# Autodesk Inventor assembly: !drivetrain
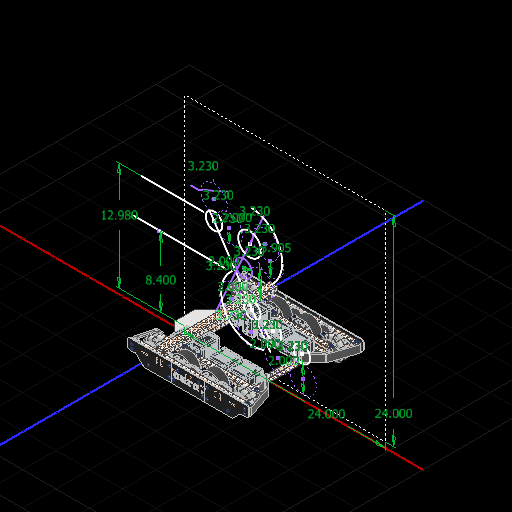
[picture p0: Inventor's stored thumbnail of the model, 512x512]
Saved by Autodesk Inventor 2025.2 (Build 292293000, 293)
## iProperties
Created: 2025-11-15
Part Number: !drivetrain
Document SubType Name: Assembly
Designer: cloudy
Mass: 2833.59 g
Surface Area: 13149.9 cm^2
Volume: 1429.88 cm^3
Density: 1.9817 g/cm^3
Author: cloudy
## Documents named in this file (40)
- C:\Users\cloudy\Documents\AURA_CAD\24\Drivetrain\!drivetrain.iam
- C:\Users\cloudy\Documents\AURA_CAD\24\Drivetrain\Wheels\Omni\2.75\2.75 Omni Assembly.iam
- C:\Users\cloudy\Documents\AURA_CAD\!lib\Structure\C Channel\Aluminum 1x2x1\Alu C 1x2x1x28.ipt
- C:\Users\cloudy\Documents\AURA_CAD\!lib\Structure\Hardware\Screw Steel - Star\SScrew Star Smooth 2.000.ipt
- C:\Users\cloudy\Documents\AURA_CAD\!lib\Structure\Hardware\Nut Keps.ipt
- C:\Users\cloudy\Documents\AURA_CAD\24\Drivetrain\Gears\26t_no_screwholes.ipt
- C:\Users\cloudy\Documents\AURA_CAD\!lib\Electronics\Motors with Screws\AluM-StarS.iam
- C:\Users\cloudy\Documents\AURA_CAD\24\Drivetrain\bearing_2 long.ipt
- C:\Users\cloudy\Documents\AURA_CAD\!lib\Motion\Spacers\Spacer Nylon .500 OD\NSpacer White .500 OD x .125.ipt
- C:\Users\cloudy\Documents\AURA_CAD\!lib\Motion\Spacers\Spacer Nylon .375 OD\NSpacer .375 OD x .500.ipt
- C:\Users\cloudy\Documents\AURA_CAD\!lib\Motion\Spacers\Spacer Nylon .375 OD\NSpacer .375 OD x .250.ipt
- C:\Users\cloudy\Documents\AURA_CAD\!lib\Motion\Shaft LS\Bearing Flat - Drilled.ipt
- C:\Users\cloudy\Documents\AURA_CAD\!lib\Motion\Shaft LS\Shaft Collar Metal\Shaft Collar No Screw.iam
- C:\Users\cloudy\Documents\AURA_CAD\!lib\Motion\Spacers\Spacer Nylon .375 OD\NSpacer .375 OD x .375.ipt
- C:\Users\cloudy\Documents\AURA_CAD\!lib\Structure\C Channel\Aluminum 1x3x1 Half\Alu C Half 1x3x1x3.ipt
- C:\Users\cloudy\Documents\AURA_CAD\24\Drivetrain\Wheels\Traction\traction.iam
- C:\Users\cloudy\Documents\AURA_CAD\!lib\Structure\Hardware\Nut Nylock.ipt
- C:\Users\cloudy\Documents\AURA_CAD\24\ziptie.ipt
- C:\Users\cloudy\Documents\AURA_CAD\!lib\Motion\Shaft LS\Shaft LS Capped\Shaft LS Capped 3.0.ipt
- C:\Users\cloudy\Documents\AURA_CAD\!lib\Structure\Hardware\Screw Steel - Star\SScrew Star Smooth .375.ipt
- C:\Users\cloudy\Documents\AURA_CAD\!lib\Structure\Hardware\Screw Steel - Star\SScrew Star Threaded .500.ipt
- C:\Users\cloudy\Documents\AURA_CAD\24\Drivetrain\funnel.ipt
- C:\Users\cloudy\Documents\AURA_CAD\!lib\Structure\C Channel\Aluminum 1x3x1 Half Thick Cut\Alu C Half Thick 1x3x1x20.ipt
- C:\Users\cloudy\Documents\AURA_CAD\!lib\Motion\Spacers\Spacer Nylon .375 OD\NSpacer .375 OD x .125.ipt
- C:\Users\cloudy\Documents\AURA_CAD\24\funnelFront.ipt
- C:\Users\cloudy\Documents\AURA_CAD\24\plate.ipt
- C:\Users\cloudy\Documents\AURA_CAD\!lib\Structure\Hardware\Screw Steel - Star\SScrew Star Smooth 1.250.ipt
- C:\Users\cloudy\Documents\GitHub\aura-cad\!lib\Structure\Hardware\Screw Steel - Star.ipt
- C:\Users\cloudy\Documents\GitHub\aura-cad\!lib\Electronics\Motors with Screws.iam
- C:\Users\cloudy\Documents\GitHub\aura-cad\!lib\Motion\Spacers\Spacer Nylon .500 OD.ipt
- C:\Users\cloudy\Documents\GitHub\aura-cad\!lib\Motion\Spacers\Spacer Nylon .375 OD.ipt
- C:\Users\cloudy\Documents\GitHub\aura-cad\!lib\Motion\Shaft LS\Shaft Collar Metal.iam
- C:\Users\cloudy\Documents\GitHub\aura-cad\!lib\Motion\Shaft LS\Shaft LS Capped.ipt
- C:\Users\cloudy\Documents\AURA_CAD\!lib\Structure\C Channel\Aluminum 1x2x1\Alu C 1x2x1x27.ipt
- C:\Users\cloudy\Documents\AURA_CAD\!lib\Structure\C Channel\Aluminum 1x3x1 Half\Alu C Half 1x3x1x27.ipt
- C:\Users\cloudy\Documents\AURA_CAD\!lib\Structure\C Channel\Aluminum 1x2x1\Alu C 1x2x1x19.ipt
- C:\Users\cloudy\Documents\AURA_CAD\24\back_funnel.ipt
- C:\Users\cloudy\Documents\AURA_CAD\!lib\Structure\C Channel\Aluminum 1x2x1\Alu C 1x2x1x25.ipt
- C:\Users\cloudy\Documents\AURA_CAD\24\wedge.ipt
- C:\Users\cloudy\Documents\AURA_CAD\!lib\Miscellaneous\iw_metal_02.bmp
## Components (186 placed, 32 different names)
1. Alu C 1x2x1x25:2 — Insert:10, Insert:19, Insert:20, Insert:36, Insert:40, Mate:22, Mate:23, Insert:41, Insert:42, Insert:43, Insert:47, Mate:24, Insert:51, Insert:90, Mate:37, Mate:38, Insert:117, Insert:122, Insert:123, Insert:163, Insert:164, Insert:165, Mate:92, Insert:313, Insert:315, Mate:100, Insert:337, Mate:102, Insert:338
2. SScrew Star Smooth 2.000:1 — Insert:10, Mate:26
3. 2.75 Omni Assembly:5 [sub-assembly] — Insert:46
4. SScrew Star Smooth 2.000:2 — Insert:20
5. SScrew Star Smooth 2.000:3 — Insert:19
6. 2.75 Omni Assembly:7 [sub-assembly] — Insert:44
7. 26t_no_screwholes:1 — Insert:52, Insert:56
8. 26t_no_screwholes:2 — Insert:53, Insert:55
9. 26t_no_screwholes:3 — Insert:54, Insert:57
10. Alu C 1x2x1x28:3 — Mate:26, Insert:52, Insert:53, Insert:54, Insert:58, Insert:59, Insert:60, Mate:27, Mate:28, Mate:29, Insert:61, Mate:30, Insert:62, Insert:63, Insert:64, Mate:31, Mate:32, Mate:33, Insert:124, Insert:125, Insert:127, Insert:128, Insert:129, Insert:130, Insert:131, Insert:132, Insert:133, Insert:134, Mate:49, Mate:50, Mate:51, Mate:52, Mate:53, Mate:54, Mate:55, Mate:56, Mate:57, Mate:58, Insert:135, Insert:136, Insert:137, Insert:138, Insert:283, Insert:284, Mate:93, Insert:294, Mate:95, Insert:297, Mate:97, Insert:314, Insert:316, Insert:335
11. AluM-StarS:1 [sub-assembly] — Insert:36, Mate:22
12. AluM-StarS:2 [sub-assembly] — Insert:40, Mate:23
13. AluM-StarS:3 [sub-assembly] — Insert:47, Mate:24
14. Nut Keps:1 — Insert:41, Insert:44
15. Nut Keps:2 — Insert:42, Insert:111
16. Nut Keps:3 — Insert:43, Insert:46
17. NSpacer White .500 OD x .125:2 — Insert:51
18. NSpacer .375 OD x .250:2 — Insert:56
19. NSpacer .375 OD x .250:3 — Insert:55
20. NSpacer .375 OD x .250:4 — Insert:57
21. bearing_2 long:3 — Insert:59, Mate:28
22. bearing_2 long:4 — Insert:61, Mate:30, Insert:112
23. bearing_2 long:5 — Insert:58, Mate:29
24. bearing_2 long:6 — Insert:60, Mate:27
25. Bearing Flat - Drilled:1 — Insert:62, Mate:33
26. Bearing Flat - Drilled:2 — Insert:64, Mate:31
27. Bearing Flat - Drilled:3 — Insert:63, Mate:32
28. Alu C Half 1x3x1x3:1 — Insert:90, Mate:37, Insert:91, Insert:147, Insert:148
29. AluM-StarS:7 [sub-assembly] — Insert:91, Mate:38
30. traction:1 [sub-assembly] — Insert:113
31. traction:2 [sub-assembly] — Insert:111, Insert:114
32. NSpacer .375 OD x .250:9 — Insert:112, Insert:113
33. Nut Nylock:1 — Insert:114
34. NSpacer .375 OD x .500:10 — Insert:116, Insert:117
35. NSpacer .375 OD x .375:11 — Insert:115
36. Shaft Collar No Screw:6 [sub-assembly] — Insert:115, Insert:116
37. NSpacer .375 OD x .500:12 — Insert:122
38. NSpacer .375 OD x .375:13
39. Shaft Collar No Screw:7 [sub-assembly]
40. NSpacer .375 OD x .500:14 — Insert:123
41. NSpacer .375 OD x .375:15
42. Shaft Collar No Screw:8 [sub-assembly]
43. ziptie:1 — Insert:125, Mate:56
44. ziptie:2 — Insert:127, Mate:57
45. ziptie:3 — Insert:128, Mate:55
46. ziptie:4 — Insert:124, Mate:58
47. ziptie:5 — Insert:129, Mate:53
48. ziptie:6 — Insert:130, Mate:54
49. ziptie:7 — Insert:131, Mate:52
50. ziptie:8 — Insert:133, Mate:50
51. ziptie:9 — Insert:132, Mate:51
52. ziptie:10 — Insert:134, Mate:49
53. Shaft LS Capped 3.0:1 — Insert:135
54. Shaft LS Capped 3.0:2 — Insert:136
55. Shaft LS Capped 3.0:3 — Insert:137
56. Shaft LS Capped 3.0:4 — Insert:138
57. NSpacer White .500 OD x .125:4
58. Nut Keps:5 — Insert:147
59. Nut Keps:6 — Insert:148
60. Nut Keps:7
61. SScrew Star Threaded .500:7 — Insert:164
62. SScrew Star Smooth .375:8 — Insert:163
63. SScrew Star Smooth .375:10 — Insert:165
64. Alu C 1x2x1x25:1 — Insert:172, Insert:173, Insert:174, Mate:60, Insert:178, Mate:61, Insert:179, Mate:62, Insert:180, Insert:182, Insert:183, Insert:185, Insert:186, Mate:71, Insert:204, Mate:72, Insert:213, Insert:216, Insert:219, Insert:252, Insert:253, Insert:263, Mate:91, Insert:317, Insert:319, Mate:99, Mate:100
65. SScrew Star Smooth 2.000:17 — Insert:172, Mate:59
66. 2.75 Omni Assembly:8 [sub-assembly] — Insert:184
67. SScrew Star Smooth 2.000:18 — Insert:173
68. SScrew Star Smooth 2.000:19 — Insert:174
69. 2.75 Omni Assembly:9 [sub-assembly] — Insert:181
70. 26t_no_screwholes:4 — Insert:177, Insert:187
71. 26t_no_screwholes:5 — Insert:176, Insert:188
72. 26t_no_screwholes:6 — Insert:175, Insert:189
73. Alu C 1x2x1x28:4 — Insert:175, Insert:176, Insert:177, Mate:59, Mate:63, Insert:190, Mate:64, Insert:191, Mate:65, Insert:192, Mate:66, Insert:193, Mate:67, Insert:194, Mate:68, Insert:195, Mate:69, Insert:196, Mate:75, Insert:222, Mate:76, Insert:223, Mate:77, Insert:224, Mate:78, Insert:225, Mate:79, Insert:226, Mate:80, Insert:227, Mate:81, Insert:228, Mate:82, Insert:229, Mate:83, Insert:230, Mate:84, Insert:231, Insert:232, Insert:233, Insert:234, Insert:235, Insert:282, Insert:285, Mate:94, Insert:295, Insert:296, Mate:96, Mate:98, Insert:318, Insert:320, Mate:103, Insert:339
74. AluM-StarS:8 [sub-assembly] — Mate:60, Insert:178
75. AluM-StarS:9 [sub-assembly] — Mate:61, Insert:179
76. AluM-StarS:10 [sub-assembly] — Mate:62, Insert:180
77. Nut Keps:11 — Insert:181, Insert:182
78. Nut Keps:12 — Insert:183, Insert:209
79. Nut Keps:13 — Insert:184, Insert:185
80. NSpacer White .500 OD x .125:6 — Insert:186
81. NSpacer .375 OD x .250:23 — Insert:187
82. NSpacer .375 OD x .250:24 — Insert:188
83. NSpacer .375 OD x .250:25 — Insert:189
84. bearing_2 long:7 — Mate:63, Insert:190
85. bearing_2 long:8 — Mate:64, Insert:191, Insert:211
86. bearing_2 long:9 — Mate:65, Insert:192
87. bearing_2 long:10 — Mate:66, Insert:193
88. Bearing Flat - Drilled:4 — Mate:67, Insert:194
89. Bearing Flat - Drilled:5 — Mate:68, Insert:195
90. Bearing Flat - Drilled:6 — Mate:69, Insert:196
91. Alu C Half 1x3x1x3:2 — Mate:71, Insert:204, Insert:205, Insert:242, Insert:243
92. AluM-StarS:11 [sub-assembly] — Mate:72, Insert:205
93. traction:3 [sub-assembly] — Insert:210
94. traction:4 [sub-assembly] — Insert:209, Insert:212
95. NSpacer .375 OD x .250:30 — Insert:210, Insert:211
96. Nut Nylock:6 — Insert:212
97. NSpacer .375 OD x .500:31 — Insert:213, Insert:214
98. NSpacer .375 OD x .375:32 — Insert:215
99. Shaft Collar No Screw:12 [sub-assembly] — Insert:214, Insert:215
100. NSpacer .375 OD x .500:33 — Insert:216, Insert:217
101. NSpacer .375 OD x .375:34 — Insert:218
102. Shaft Collar No Screw:13 [sub-assembly] — Insert:217, Insert:218
103. NSpacer .375 OD x .500:35 — Insert:219, Insert:220
104. NSpacer .375 OD x .375:36 — Insert:221
105. Shaft Collar No Screw:14 [sub-assembly] — Insert:220, Insert:221
106. ziptie:11 — Mate:75, Insert:222
107. ziptie:12 — Mate:76, Insert:223
108. ziptie:13 — Mate:77, Insert:224
109. ziptie:14 — Mate:78, Insert:225
110. ziptie:15 — Mate:79, Insert:226
111. ziptie:16 — Mate:80, Insert:227
112. ziptie:17 — Mate:81, Insert:228
113. ziptie:18 — Mate:82, Insert:229
114. ziptie:19 — Mate:83, Insert:230
115. ziptie:20 — Mate:84, Insert:231
116. Shaft LS Capped 3.0:5 — Insert:232
117. Shaft LS Capped 3.0:6 — Insert:233
118. Shaft LS Capped 3.0:7 — Insert:234
119. Shaft LS Capped 3.0:8 — Insert:235
120. NSpacer White .500 OD x .125:8
121. Nut Keps:15 — Insert:242
122. Nut Keps:16 — Insert:243
123. Nut Keps:17
124. SScrew Star Smooth .375:24 — Insert:252
125. SScrew Star Smooth .375:25 — Insert:253
126. SScrew Star Threaded .500:32 — Insert:263
127. funnel:2 — Insert:282, Mate:91
128. funnel:3 — Insert:283, Mate:92
129. Alu C Half Thick 1x3x1x20:1 — Insert:284, Mate:93, Insert:287, Insert:289, Flush:1, Mate:101
130. Alu C Half Thick 1x3x1x20:2 — Insert:285, Mate:94, Insert:291, Insert:293, Insert:298, Insert:336
131. NSpacer .375 OD x .500:44 — Insert:286, Insert:287
132. NSpacer .375 OD x .125:45 — Insert:286
133. NSpacer .375 OD x .500:46 — Insert:289
134. NSpacer .375 OD x .125:47
135. NSpacer .375 OD x .500:48 — Insert:291
136. NSpacer .375 OD x .125:49
137. NSpacer .375 OD x .500:50 — Insert:293
138. NSpacer .375 OD x .125:51
139. funnelFront:1 — Insert:295, Insert:321, Insert:322, Insert:323, Insert:324, Insert:325
140. funnelFront:2 — Insert:294, Mate:95, Insert:299, Insert:300, Insert:301, Insert:302, Insert:303, Flush:2, Mate:104, Mate:105
141. funnelFront:3 — Insert:296, Mate:96, Insert:330, Insert:331, Insert:332, Insert:333, Insert:334
142. funnelFront:4 — Insert:297, Mate:97, Insert:308, Insert:309, Insert:310, Insert:311, Insert:312
143. plate:1 — Flush:1, Insert:304, Insert:305, Insert:306, Insert:307, Flush:2, Mate:104, Mate:105
144. plate:2 — Insert:298, Mate:98, Insert:326, Insert:327, Insert:328, Insert:329
145. SScrew Star Smooth .375:40 — Insert:301
146. SScrew Star Smooth .375:41 — Insert:302
147. SScrew Star Smooth .375:42 — Insert:300
148. SScrew Star Smooth .375:43 — Insert:303
149. SScrew Star Smooth .375:44 — Insert:299
150. SScrew Star Smooth .375:45 — Insert:310
151. SScrew Star Smooth .375:46 — Insert:311
152. SScrew Star Smooth .375:47 — Insert:309
153. SScrew Star Smooth .375:48 — Insert:312
154. SScrew Star Smooth .375:49 — Insert:307
155. SScrew Star Smooth .375:50 — Insert:308
156. SScrew Star Smooth .375:51 — Insert:306
157. SScrew Star Smooth .375:52 — Insert:304
158. SScrew Star Smooth .375:53 — Insert:305
159. Nut Nylock:16 — Insert:315
160. SScrew Star Smooth 1.250:54 — Insert:314
161. Nut Nylock:17 — Insert:316
162. SScrew Star Smooth 1.250:55 — Insert:313
163. Nut Nylock:18 — Insert:319
164. SScrew Star Smooth 1.250:56 — Insert:318
165. Nut Nylock:19 — Insert:320
166. SScrew Star Smooth 1.250:57 — Insert:317
167. SScrew Star Smooth .375:58 — Insert:321
168. SScrew Star Smooth .375:59 — Insert:325
169. SScrew Star Smooth .375:60 — Insert:322
170. SScrew Star Smooth .375:61 — Insert:324, Mate:103
171. SScrew Star Smooth .375:62 — Insert:323
172. SScrew Star Smooth .375:63 — Insert:333
173. SScrew Star Smooth .375:64 — Insert:329
174. SScrew Star Smooth .375:65 — Insert:330
175. SScrew Star Smooth .375:66 — Insert:328
176. SScrew Star Smooth .375:67 — Insert:334
177. SScrew Star Smooth .375:68 — Insert:332
178. SScrew Star Smooth .375:69 — Insert:331
179. SScrew Star Smooth .375:70 — Insert:326
180. SScrew Star Smooth .375:71 — Insert:327
181. Alu C 1x2x1x27:1 — Insert:335, Mate:99
182. Alu C Half 1x3x1x27:1 — Insert:336, Mate:101
183. Alu C 1x2x1x19:1 — Insert:337, Mate:102, Flush:3
184. back_funnel:1 — Insert:338
185. back_funnel:2 — Insert:339
186. wedge:1 — Flush:3
## Relationships (240: Insert 176, Mate 61, Flush 3)
- Insert:10: Alu C 1x2x1x25:2 ↔ SScrew Star Smooth 2.000:1
- Insert:19: Alu C 1x2x1x25:2 ↔ SScrew Star Smooth 2.000:3
- Insert:20: Alu C 1x2x1x25:2 ↔ SScrew Star Smooth 2.000:2
- Insert:36: Alu C 1x2x1x25:2 ↔ AluM-StarS:1
- Insert:40: Alu C 1x2x1x25:2 ↔ AluM-StarS:2
- Mate:22: Alu C 1x2x1x25:2 ↔ AluM-StarS:1
- Mate:23: Alu C 1x2x1x25:2 ↔ AluM-StarS:2
- Insert:41: Alu C 1x2x1x25:2 ↔ Nut Keps:1
- Insert:42: Alu C 1x2x1x25:2 ↔ Nut Keps:2
- Insert:43: Alu C 1x2x1x25:2 ↔ Nut Keps:3
- Insert:44 (0.7937 mm): 2.75 Omni Assembly:7 ↔ Nut Keps:1
- Insert:46 (0.7937 mm): 2.75 Omni Assembly:5 ↔ Nut Keps:3
- Insert:47: Alu C 1x2x1x25:2 ↔ AluM-StarS:3
- Mate:24: Alu C 1x2x1x25:2 ↔ AluM-StarS:3
- Insert:51: Alu C 1x2x1x25:2 ↔ NSpacer White .500 OD x .125:2
- Mate:26: SScrew Star Smooth 2.000:1 ↔ Alu C 1x2x1x28:3
- Insert:52 (13.4938 mm): 26t_no_screwholes:1 ↔ Alu C 1x2x1x28:3
- Insert:53 (13.4938 mm): 26t_no_screwholes:2 ↔ Alu C 1x2x1x28:3
- Insert:54 (13.4938 mm): 26t_no_screwholes:3 ↔ Alu C 1x2x1x28:3
- Insert:55: 26t_no_screwholes:2 ↔ NSpacer .375 OD x .250:3
- Insert:56: 26t_no_screwholes:1 ↔ NSpacer .375 OD x .250:2
- Insert:57: 26t_no_screwholes:3 ↔ NSpacer .375 OD x .250:4
- Insert:58: Alu C 1x2x1x28:3 ↔ bearing_2 long:5
- Insert:59: Alu C 1x2x1x28:3 ↔ bearing_2 long:3
- Insert:60: Alu C 1x2x1x28:3 ↔ bearing_2 long:6
- Mate:27: Alu C 1x2x1x28:3 ↔ bearing_2 long:6
- Mate:28: Alu C 1x2x1x28:3 ↔ bearing_2 long:3
- Mate:29: Alu C 1x2x1x28:3 ↔ bearing_2 long:5
- Insert:61: Alu C 1x2x1x28:3 ↔ bearing_2 long:4
- Mate:30: Alu C 1x2x1x28:3 ↔ bearing_2 long:4
- Insert:62: Alu C 1x2x1x28:3 ↔ Bearing Flat - Drilled:1
- Insert:63: Alu C 1x2x1x28:3 ↔ Bearing Flat - Drilled:3
- Insert:64: Alu C 1x2x1x28:3 ↔ Bearing Flat - Drilled:2
- Mate:31: Alu C 1x2x1x28:3 ↔ Bearing Flat - Drilled:2
- Mate:32: Alu C 1x2x1x28:3 ↔ Bearing Flat - Drilled:3
- Mate:33: Alu C 1x2x1x28:3 ↔ Bearing Flat - Drilled:1
- Insert:90: Alu C 1x2x1x25:2 ↔ Alu C Half 1x3x1x3:1
- Mate:37: Alu C 1x2x1x25:2 ↔ Alu C Half 1x3x1x3:1
- Insert:91: Alu C Half 1x3x1x3:1 ↔ AluM-StarS:7
- Mate:38: Alu C 1x2x1x25:2 ↔ AluM-StarS:7
- Insert:111: Nut Keps:2 ↔ traction:2
- Insert:112 (0.7937 mm): bearing_2 long:4 ↔ NSpacer .375 OD x .250:9
- Insert:113: traction:1 ↔ NSpacer .375 OD x .250:9
- Insert:114: traction:2 ↔ Nut Nylock:1
- Insert:115: NSpacer .375 OD x .375:11 ↔ Shaft Collar No Screw:6
- Insert:116: NSpacer .375 OD x .500:10 ↔ Shaft Collar No Screw:6
- Insert:117 (1.016 mm): Alu C 1x2x1x25:2 ↔ NSpacer .375 OD x .500:10
- [Insert]: NSpacer .375 OD x .375:13 ↔ Shaft Collar No Screw:7
- [Insert]: NSpacer .375 OD x .500:12 ↔ Shaft Collar No Screw:7
- [Insert]: NSpacer .375 OD x .375:15 ↔ Shaft Collar No Screw:8
- [Insert]: NSpacer .375 OD x .500:14 ↔ Shaft Collar No Screw:8
- Insert:122 (1.016 mm): Alu C 1x2x1x25:2 ↔ NSpacer .375 OD x .500:12
- Insert:123 (1.016 mm): Alu C 1x2x1x25:2 ↔ NSpacer .375 OD x .500:14
- Insert:124: Alu C 1x2x1x28:3 ↔ ziptie:4
- Insert:125: Alu C 1x2x1x28:3 ↔ ziptie:1
- Insert:127: Alu C 1x2x1x28:3 ↔ ziptie:2
- Insert:128: Alu C 1x2x1x28:3 ↔ ziptie:3
- Insert:129: Alu C 1x2x1x28:3 ↔ ziptie:5
- Insert:130: Alu C 1x2x1x28:3 ↔ ziptie:6
- Insert:131: Alu C 1x2x1x28:3 ↔ ziptie:7
- Insert:132: Alu C 1x2x1x28:3 ↔ ziptie:9
- Insert:133: Alu C 1x2x1x28:3 ↔ ziptie:8
- Insert:134: Alu C 1x2x1x28:3 ↔ ziptie:10
- Mate:49: Alu C 1x2x1x28:3 ↔ ziptie:10
- Mate:50: Alu C 1x2x1x28:3 ↔ ziptie:8
- Mate:51: Alu C 1x2x1x28:3 ↔ ziptie:9
- Mate:52: Alu C 1x2x1x28:3 ↔ ziptie:7
- Mate:53: Alu C 1x2x1x28:3 ↔ ziptie:5
- Mate:54: Alu C 1x2x1x28:3 ↔ ziptie:6
- Mate:55: Alu C 1x2x1x28:3 ↔ ziptie:3
- Mate:56: Alu C 1x2x1x28:3 ↔ ziptie:1
- Mate:57: Alu C 1x2x1x28:3 ↔ ziptie:2
- Mate:58: Alu C 1x2x1x28:3 ↔ ziptie:4
- Insert:135: Alu C 1x2x1x28:3 ↔ Shaft LS Capped 3.0:1
- Insert:136: Alu C 1x2x1x28:3 ↔ Shaft LS Capped 3.0:2
- Insert:137: Alu C 1x2x1x28:3 ↔ Shaft LS Capped 3.0:3
- Insert:138: Alu C 1x2x1x28:3 ↔ Shaft LS Capped 3.0:4
- Insert:147: Alu C Half 1x3x1x3:1 ↔ Nut Keps:5
- Insert:148: Alu C Half 1x3x1x3:1 ↔ Nut Keps:6
- Insert:163: Alu C 1x2x1x25:2 ↔ SScrew Star Smooth .375:8
- Insert:164: Alu C 1x2x1x25:2 ↔ SScrew Star Threaded .500:7
- Insert:165: Alu C 1x2x1x25:2 ↔ SScrew Star Smooth .375:10
- Insert:172: Alu C 1x2x1x25:1 ↔ SScrew Star Smooth 2.000:17
- Insert:173: Alu C 1x2x1x25:1 ↔ SScrew Star Smooth 2.000:18
- Insert:174: Alu C 1x2x1x25:1 ↔ SScrew Star Smooth 2.000:19
- Insert:175 (13.4938 mm): 26t_no_screwholes:6 ↔ Alu C 1x2x1x28:4
- Insert:176 (13.4938 mm): 26t_no_screwholes:5 ↔ Alu C 1x2x1x28:4
- Insert:177 (13.4938 mm): 26t_no_screwholes:4 ↔ Alu C 1x2x1x28:4
- Mate:59: SScrew Star Smooth 2.000:17 ↔ Alu C 1x2x1x28:4
- Mate:60: Alu C 1x2x1x25:1 ↔ AluM-StarS:8
- Insert:178: Alu C 1x2x1x25:1 ↔ AluM-StarS:8
- Mate:61: Alu C 1x2x1x25:1 ↔ AluM-StarS:9
- Insert:179: Alu C 1x2x1x25:1 ↔ AluM-StarS:9
- Mate:62: Alu C 1x2x1x25:1 ↔ AluM-StarS:10
- Insert:180: Alu C 1x2x1x25:1 ↔ AluM-StarS:10
- Insert:181 (0.7937 mm): 2.75 Omni Assembly:9 ↔ Nut Keps:11
- Insert:182: Alu C 1x2x1x25:1 ↔ Nut Keps:11
- Insert:183: Alu C 1x2x1x25:1 ↔ Nut Keps:12
- Insert:184 (0.7937 mm): 2.75 Omni Assembly:8 ↔ Nut Keps:13
- Insert:185: Alu C 1x2x1x25:1 ↔ Nut Keps:13
- Insert:186: Alu C 1x2x1x25:1 ↔ NSpacer White .500 OD x .125:6
- Insert:187: 26t_no_screwholes:4 ↔ NSpacer .375 OD x .250:23
- Insert:188: 26t_no_screwholes:5 ↔ NSpacer .375 OD x .250:24
- Insert:189: 26t_no_screwholes:6 ↔ NSpacer .375 OD x .250:25
- Mate:63: Alu C 1x2x1x28:4 ↔ bearing_2 long:7
- Insert:190: Alu C 1x2x1x28:4 ↔ bearing_2 long:7
- Mate:64: Alu C 1x2x1x28:4 ↔ bearing_2 long:8
- Insert:191: Alu C 1x2x1x28:4 ↔ bearing_2 long:8
- Mate:65: Alu C 1x2x1x28:4 ↔ bearing_2 long:9
- Insert:192: Alu C 1x2x1x28:4 ↔ bearing_2 long:9
- Mate:66: Alu C 1x2x1x28:4 ↔ bearing_2 long:10
- Insert:193: Alu C 1x2x1x28:4 ↔ bearing_2 long:10
- Mate:67: Alu C 1x2x1x28:4 ↔ Bearing Flat - Drilled:4
- Insert:194: Alu C 1x2x1x28:4 ↔ Bearing Flat - Drilled:4
- Mate:68: Alu C 1x2x1x28:4 ↔ Bearing Flat - Drilled:5
- Insert:195: Alu C 1x2x1x28:4 ↔ Bearing Flat - Drilled:5
- Mate:69: Alu C 1x2x1x28:4 ↔ Bearing Flat - Drilled:6
- Insert:196: Alu C 1x2x1x28:4 ↔ Bearing Flat - Drilled:6
- Mate:71: Alu C 1x2x1x25:1 ↔ Alu C Half 1x3x1x3:2
- Insert:204: Alu C 1x2x1x25:1 ↔ Alu C Half 1x3x1x3:2
- Mate:72: Alu C 1x2x1x25:1 ↔ AluM-StarS:11
- Insert:205: Alu C Half 1x3x1x3:2 ↔ AluM-StarS:11
- Insert:209: Nut Keps:12 ↔ traction:4
- Insert:210: traction:3 ↔ NSpacer .375 OD x .250:30
- Insert:211 (0.7937 mm): bearing_2 long:8 ↔ NSpacer .375 OD x .250:30
- Insert:212: traction:4 ↔ Nut Nylock:6
- Insert:213 (1.016 mm): Alu C 1x2x1x25:1 ↔ NSpacer .375 OD x .500:31
- Insert:214: NSpacer .375 OD x .500:31 ↔ Shaft Collar No Screw:12
- Insert:215: NSpacer .375 OD x .375:32 ↔ Shaft Collar No Screw:12
- Insert:216 (1.016 mm): Alu C 1x2x1x25:1 ↔ NSpacer .375 OD x .500:33
- Insert:217: NSpacer .375 OD x .500:33 ↔ Shaft Collar No Screw:13
- Insert:218: NSpacer .375 OD x .375:34 ↔ Shaft Collar No Screw:13
- Insert:219 (1.016 mm): Alu C 1x2x1x25:1 ↔ NSpacer .375 OD x .500:35
- Insert:220: NSpacer .375 OD x .500:35 ↔ Shaft Collar No Screw:14
- Insert:221: NSpacer .375 OD x .375:36 ↔ Shaft Collar No Screw:14
- Mate:75: Alu C 1x2x1x28:4 ↔ ziptie:11
- Insert:222: Alu C 1x2x1x28:4 ↔ ziptie:11
- Mate:76: Alu C 1x2x1x28:4 ↔ ziptie:12
- Insert:223: Alu C 1x2x1x28:4 ↔ ziptie:12
- Mate:77: Alu C 1x2x1x28:4 ↔ ziptie:13
- Insert:224: Alu C 1x2x1x28:4 ↔ ziptie:13
- Mate:78: Alu C 1x2x1x28:4 ↔ ziptie:14
- Insert:225: Alu C 1x2x1x28:4 ↔ ziptie:14
- Mate:79: Alu C 1x2x1x28:4 ↔ ziptie:15
- Insert:226: Alu C 1x2x1x28:4 ↔ ziptie:15
- Mate:80: Alu C 1x2x1x28:4 ↔ ziptie:16
- Insert:227: Alu C 1x2x1x28:4 ↔ ziptie:16
- Mate:81: Alu C 1x2x1x28:4 ↔ ziptie:17
- Insert:228: Alu C 1x2x1x28:4 ↔ ziptie:17
- Mate:82: Alu C 1x2x1x28:4 ↔ ziptie:18
- Insert:229: Alu C 1x2x1x28:4 ↔ ziptie:18
- Mate:83: Alu C 1x2x1x28:4 ↔ ziptie:19
- Insert:230: Alu C 1x2x1x28:4 ↔ ziptie:19
- Mate:84: Alu C 1x2x1x28:4 ↔ ziptie:20
- Insert:231: Alu C 1x2x1x28:4 ↔ ziptie:20
- Insert:232: Alu C 1x2x1x28:4 ↔ Shaft LS Capped 3.0:5
- Insert:233: Alu C 1x2x1x28:4 ↔ Shaft LS Capped 3.0:6
- Insert:234: Alu C 1x2x1x28:4 ↔ Shaft LS Capped 3.0:7
- Insert:235: Alu C 1x2x1x28:4 ↔ Shaft LS Capped 3.0:8
- Insert:242: Alu C Half 1x3x1x3:2 ↔ Nut Keps:15
- Insert:243: Alu C Half 1x3x1x3:2 ↔ Nut Keps:16
- Insert:252: Alu C 1x2x1x25:1 ↔ SScrew Star Smooth .375:24
- Insert:253: Alu C 1x2x1x25:1 ↔ SScrew Star Smooth .375:25
- Insert:263: Alu C 1x2x1x25:1 ↔ SScrew Star Threaded .500:32
- Insert:282: Alu C 1x2x1x28:4 ↔ funnel:2
- Mate:91: Alu C 1x2x1x25:1 ↔ funnel:2
- Insert:283: Alu C 1x2x1x28:3 ↔ funnel:3
- Mate:92: Alu C 1x2x1x25:2 ↔ funnel:3
- Insert:284 (15.875 mm): Alu C 1x2x1x28:3 ↔ Alu C Half Thick 1x3x1x20:1
- Mate:93: Alu C 1x2x1x28:3 ↔ Alu C Half Thick 1x3x1x20:1
- Insert:285 (15.875 mm): Alu C 1x2x1x28:4 ↔ Alu C Half Thick 1x3x1x20:2
- Mate:94: Alu C 1x2x1x28:4 ↔ Alu C Half Thick 1x3x1x20:2
- Insert:286: NSpacer .375 OD x .500:44 ↔ NSpacer .375 OD x .125:45
- Insert:287: Alu C Half Thick 1x3x1x20:1 ↔ NSpacer .375 OD x .500:44
- [Insert]: NSpacer .375 OD x .500:46 ↔ NSpacer .375 OD x .125:47
- Insert:289: Alu C Half Thick 1x3x1x20:1 ↔ NSpacer .375 OD x .500:46
- [Insert]: NSpacer .375 OD x .500:48 ↔ NSpacer .375 OD x .125:49
- Insert:291: Alu C Half Thick 1x3x1x20:2 ↔ NSpacer .375 OD x .500:48
- [Insert]: NSpacer .375 OD x .500:50 ↔ NSpacer .375 OD x .125:51
- Insert:293: Alu C Half Thick 1x3x1x20:2 ↔ NSpacer .375 OD x .500:50
- Insert:294: Alu C 1x2x1x28:3 ↔ funnelFront:2
- Mate:95: Alu C 1x2x1x28:3 ↔ funnelFront:2
- Insert:295: Alu C 1x2x1x28:4 ↔ funnelFront:1
- Insert:296: Alu C 1x2x1x28:4 ↔ funnelFront:3
- Mate:96: Alu C 1x2x1x28:4 ↔ funnelFront:3
- Insert:297: Alu C 1x2x1x28:3 ↔ funnelFront:4
- Mate:97: Alu C 1x2x1x28:3 ↔ funnelFront:4
- Flush:1: Alu C Half Thick 1x3x1x20:1 ↔ plate:1
- Insert:298: Alu C Half Thick 1x3x1x20:2 ↔ plate:2
- Mate:98: Alu C 1x2x1x28:4 ↔ plate:2
- Insert:299: funnelFront:2 ↔ SScrew Star Smooth .375:44
- Insert:300: funnelFront:2 ↔ SScrew Star Smooth .375:42
- Insert:301: funnelFront:2 ↔ SScrew Star Smooth .375:40
- Insert:302: funnelFront:2 ↔ SScrew Star Smooth .375:41
- Insert:303: funnelFront:2 ↔ SScrew Star Smooth .375:43
- Insert:304: plate:1 ↔ SScrew Star Smooth .375:52
- Insert:305: plate:1 ↔ SScrew Star Smooth .375:53
- Insert:306: plate:1 ↔ SScrew Star Smooth .375:51
- Insert:307: plate:1 ↔ SScrew Star Smooth .375:49
- Insert:308: funnelFront:4 ↔ SScrew Star Smooth .375:50
- Insert:309: funnelFront:4 ↔ SScrew Star Smooth .375:47
- Insert:310: funnelFront:4 ↔ SScrew Star Smooth .375:45
- Insert:311: funnelFront:4 ↔ SScrew Star Smooth .375:46
- Insert:312: funnelFront:4 ↔ SScrew Star Smooth .375:48
- Insert:313: Alu C 1x2x1x25:2 ↔ SScrew Star Smooth 1.250:55
- Insert:314: Alu C 1x2x1x28:3 ↔ SScrew Star Smooth 1.250:54
- Insert:315: Alu C 1x2x1x25:2 ↔ Nut Nylock:16
- Insert:316: Alu C 1x2x1x28:3 ↔ Nut Nylock:17
- Insert:317: Alu C 1x2x1x25:1 ↔ SScrew Star Smooth 1.250:57
- Insert:318: Alu C 1x2x1x28:4 ↔ SScrew Star Smooth 1.250:56
- Insert:319: Alu C 1x2x1x25:1 ↔ Nut Nylock:18
- Insert:320: Alu C 1x2x1x28:4 ↔ Nut Nylock:19
- Insert:321: funnelFront:1 ↔ SScrew Star Smooth .375:58
- Insert:322: funnelFront:1 ↔ SScrew Star Smooth .375:60
- Insert:323: funnelFront:1 ↔ SScrew Star Smooth .375:62
- Insert:324: funnelFront:1 ↔ SScrew Star Smooth .375:61
- Insert:325: funnelFront:1 ↔ SScrew Star Smooth .375:59
- Insert:326: plate:2 ↔ SScrew Star Smooth .375:70
- Insert:327: plate:2 ↔ SScrew Star Smooth .375:71
- Insert:328: plate:2 ↔ SScrew Star Smooth .375:66
- Insert:329: plate:2 ↔ SScrew Star Smooth .375:64
- Insert:330: funnelFront:3 ↔ SScrew Star Smooth .375:65
- Insert:331: funnelFront:3 ↔ SScrew Star Smooth .375:69
- Insert:332: funnelFront:3 ↔ SScrew Star Smooth .375:68
- Insert:333: funnelFront:3 ↔ SScrew Star Smooth .375:63
- Insert:334: funnelFront:3 ↔ SScrew Star Smooth .375:67
- Insert:335 (19.05 mm): Alu C 1x2x1x28:3 ↔ Alu C 1x2x1x27:1
- Insert:336 (-3.5719 mm): Alu C Half Thick 1x3x1x20:2 ↔ Alu C Half 1x3x1x27:1
- Mate:99: Alu C 1x2x1x25:1 ↔ Alu C 1x2x1x27:1
- Mate:100: Alu C 1x2x1x25:2 ↔ Alu C 1x2x1x25:1
- Mate:101: Alu C Half Thick 1x3x1x20:1 ↔ Alu C Half 1x3x1x27:1
- Insert:337 (3.9688 mm): Alu C 1x2x1x25:2 ↔ Alu C 1x2x1x19:1
- Mate:102: Alu C 1x2x1x25:2 ↔ Alu C 1x2x1x19:1
- Mate:103: Alu C 1x2x1x28:4 ↔ SScrew Star Smooth .375:61
- Flush:2: funnelFront:2 ↔ plate:1
- Mate:104: funnelFront:2 ↔ plate:1
- Mate:105 (0.3969 mm): funnelFront:2 ↔ plate:1
- Insert:338: Alu C 1x2x1x25:2 ↔ back_funnel:1
- Insert:339: Alu C 1x2x1x28:4 ↔ back_funnel:2
- Flush:3: Alu C 1x2x1x19:1 ↔ wedge:1
## Named parameters: d257_d254 = 0 mm, d258_d255 = 0 mm, d259_d254 = 0 mm, d260_d255 = 0 mm, d473_d471 = 0 mm, d475_d471 = 0 mm, d477_d471 = 0 mm
